# Autodesk Inventor assembly: MainAssembly
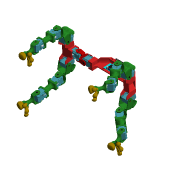
[picture p0: Inventor's stored thumbnail of the model, 180x180]
Saved by Autodesk Inventor 2016 (Build 200138000, 138)
## iProperties
Created: 2015-03-24
Part Number: MainAssembly
Document SubType Name: Assembly
Designer: Henke
Author: Henke
## Documents named in this file (10)
- G:\Study_and_Projekts\KEX_robotik\CAD\MainAssembly.iam
- G:\Study_and_Projekts\KEX_robotik\CAD\ChestConnector10Degrees.ipt
- G:\Study_and_Projekts\KEX_robotik\CAD\Leg3DOF-Front.iam
- G:\Study_and_Projekts\KEX_robotik\CAD\DCDCStepDown\Imported Components\Step Down voltage regulator LM2596\Step Down voltage regulator LM2596.ipt
- G:\Study_and_Projekts\KEX_robotik\CAD\Arduino Mega 2560\Assembly1.iam
- G:\Study_and_Projekts\KEX_robotik\CAD\RearConnector.ipt
- G:\Study_and_Projekts\KEX_robotik\CAD\SupportLeg.ipt
- G:\Study_and_Projekts\KEX_robotik\CAD\Leg3DOF-Front-Left.iam
- G:\Study_and_Projekts\KEX_robotik\CAD\RibBone.ipt
- G:\Study_and_Projekts\KEX_robotik\CAD\Spine2.iam
## Components (17 placed, 9 different names)
1. ChestConnector10Degrees:1 — Mate:4, Mate:5, Flush:1, Mate:6, Angle:1, Mate:7, Angle:2, Mate:17, Mate:18, Mate:19, Mate:20, Mate:21, Mate:22, Mate:23, Mate:24, Mate:28
2. Leg3DOF-Front:1 [sub-assembly] — Mate:4, Mate:5, Flush:1
3. Step Down voltage regulator LM2596:1 — Mate:6, Angle:1
4. Assembly1:1 [sub-assembly] — Mate:7, Angle:2
5. RearConnector:1 — Mate:25, Mate:26, Mate:27, Mate:29, Mate:30, Mate:31, Mate:32, Mate:33, Mate:34
6. SupportLeg:1 — Mate:17, Mate:18, Mate:19
7. Leg3DOF-Front-Left:1 [sub-assembly] — Mate:20, Mate:21, Mate:22
8. RibBone:1
9. RibBone:2
10. RibBone:3
11. RibBone:4
12. RibBone:5
13. RibBone:6
14. RibBone:7
15. Spine2:1 [sub-assembly] — Mate:23, Mate:24, Mate:25, Mate:26, Mate:27, Mate:28
16. Leg3DOF-Front:2 [sub-assembly] — Mate:32, Mate:33, Mate:34
17. Leg3DOF-Front-Left:2 [sub-assembly] — Mate:29, Mate:30, Mate:31
## Relationships (25: Mate 22, Angle 2, Flush 1)
- Mate:4: ChestConnector10Degrees:1 ↔ Leg3DOF-Front:1
- Mate:5: ChestConnector10Degrees:1 ↔ Leg3DOF-Front:1
- Flush:1: ChestConnector10Degrees:1 ↔ Leg3DOF-Front:1
- Mate:6: ChestConnector10Degrees:1 ↔ Step Down voltage regulator LM2596:1
- Angle:1 (0 deg): ChestConnector10Degrees:1 ↔ Step Down voltage regulator LM2596:1
- Mate:7: ChestConnector10Degrees:1 ↔ Assembly1:1
- Angle:2 (0 deg): ChestConnector10Degrees:1 ↔ Assembly1:1
- Mate:17: ChestConnector10Degrees:1 ↔ SupportLeg:1
- Mate:18: ChestConnector10Degrees:1 ↔ SupportLeg:1
- Mate:19: ChestConnector10Degrees:1 ↔ SupportLeg:1
- Mate:20: ChestConnector10Degrees:1 ↔ Leg3DOF-Front-Left:1
- Mate:21: ChestConnector10Degrees:1 ↔ Leg3DOF-Front-Left:1
- Mate:22: ChestConnector10Degrees:1 ↔ Leg3DOF-Front-Left:1
- Mate:23: ChestConnector10Degrees:1 ↔ Spine2:1
- Mate:24: ChestConnector10Degrees:1 ↔ Spine2:1
- Mate:25: RearConnector:1 ↔ Spine2:1
- Mate:26: RearConnector:1 ↔ Spine2:1
- Mate:27: RearConnector:1 ↔ Spine2:1
- Mate:28: ChestConnector10Degrees:1 ↔ Spine2:1
- Mate:29: RearConnector:1 ↔ Leg3DOF-Front-Left:2
- Mate:30: RearConnector:1 ↔ Leg3DOF-Front-Left:2
- Mate:31: RearConnector:1 ↔ Leg3DOF-Front-Left:2
- Mate:32: RearConnector:1 ↔ Leg3DOF-Front:2
- Mate:33: RearConnector:1 ↔ Leg3DOF-Front:2
- Mate:34: RearConnector:1 ↔ Leg3DOF-Front:2
